# Autodesk Inventor assembly: Stopa v1
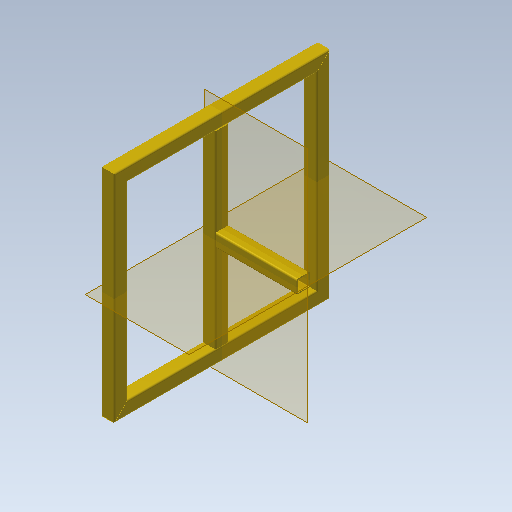
[picture p0: Inventor's stored thumbnail of the model, 512x512]
Saved by Autodesk Inventor 2021 (Build 250183000, 183)
## iProperties
Created: 2024-04-18
Part Number: Stopa v1
Document SubType Name: Assembly
Designer: Michal
Author: Michal
## Documents named in this file (5)
- C:\Users\Michal\Documents\GitHub\PNW_PhotoBoothFrame_3D\Stopa v1.iam
- C:\Users\Michal\Documents\GitHub\PNW_PhotoBoothFrame_3D\Stopa v1 profil 1.ipt
- C:\Users\Michal\Documents\GitHub\PNW_PhotoBoothFrame_3D\Stopa v1 profil 2.ipt
- C:\Users\Michal\Documents\GitHub\PNW_PhotoBoothFrame_3D\Stopa v1 profil 3.ipt
- C:\Users\Michal\Documents\GitHub\PNW_PhotoBoothFrame_3D\M8x15.ipt
## Components (8 placed, 4 different names)
1. Stopa v1 profil 1:1 — Mate:1, Flush:1, Mate:2, Mate:5, Mate:6, Mate:8, Mate:10
2. Stopa v1 profil 1:2 — Mate:1, Flush:1, Mate:2, Flush:2, Mate:3, Mate:7, Flush:4
3. Stopa v1 profil 1:3 — Flush:2, Flush:3, Mate:3, Mate:4
4. Stopa v1 profil 1:4 — Flush:3, Mate:4, Mate:5, Mate:6, Mate:9
5. Stopa v1 profil 2:1 — Mate:7, Flush:4, Mate:11, Mate:12
6. Stopa v1 profil 3:1 — Mate:12, Mate:13, Flush:5, Mate:14, Mate:15, Mate:16
7. M8x15:1 — Mate:14, Flush:6, Mate:16
8. M8x15:2 — Mate:15, Flush:6
## Relationships (22: Mate 16, Flush 6)
- Mate:1: Stopa v1 profil 1:1 ↔ Stopa v1 profil 1:2
- Flush:1: Stopa v1 profil 1:1 ↔ Stopa v1 profil 1:2
- Mate:2: Stopa v1 profil 1:1 ↔ Stopa v1 profil 1:2
- Flush:2: Stopa v1 profil 1:2 ↔ Stopa v1 profil 1:3
- Flush:3: Stopa v1 profil 1:3 ↔ Stopa v1 profil 1:4
- Mate:3: Stopa v1 profil 1:2 ↔ Stopa v1 profil 1:3
- Mate:4: Stopa v1 profil 1:3 ↔ Stopa v1 profil 1:4
- Mate:5: Stopa v1 profil 1:1 ↔ Stopa v1 profil 1:4
- Mate:6: Stopa v1 profil 1:1 ↔ Stopa v1 profil 1:4
- Mate:7: Stopa v1 profil 1:2 ↔ Stopa v1 profil 2:1
- Flush:4: Stopa v1 profil 1:2 ↔ Stopa v1 profil 2:1
- Mate:8: Stopa v1 profil 1:1
- Mate:9: Stopa v1 profil 1:4
- Mate:10: Stopa v1 profil 1:1
- Mate:11: Stopa v1 profil 2:1
- Mate:12: Stopa v1 profil 2:1 ↔ Stopa v1 profil 3:1
- Mate:13: Stopa v1 profil 3:1
- Flush:5: Stopa v1 profil 3:1
- Mate:14: Stopa v1 profil 3:1 ↔ M8x15:1
- Mate:15: Stopa v1 profil 3:1 ↔ M8x15:2
- Flush:6: M8x15:1 ↔ M8x15:2
- Mate:16 (3 mm): Stopa v1 profil 3:1 ↔ M8x15:1
